# Autodesk Inventor assembly: VERSION3-largel-upright-hook
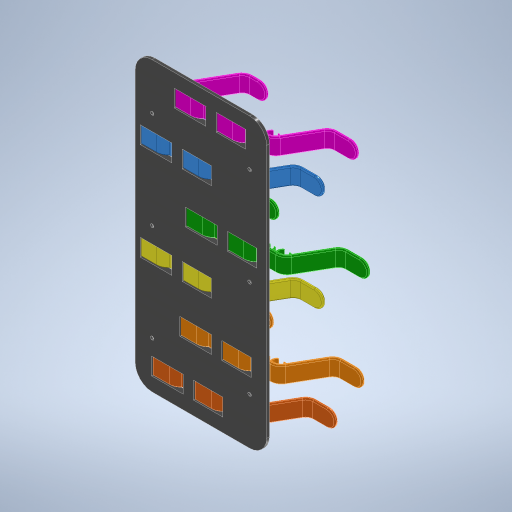
[picture p0: Inventor's stored thumbnail of the model, 512x512]
Saved by Autodesk Inventor 2024.1 (Build 281209000, 209)
## iProperties
Created: 2024-09-23
Part Number: VERSION3-largel-upright-hook
Document SubType Name: Assembly
Designer: Imogen Heard
Author: Imogen Heard
## Documents named in this file (3)
- C:\Users\iwheard\Documents\0004-CAD\3D-cad-main\cable-hanger\VERSION3-largel-upright-hook.iam
- C:\Users\iwheard\Documents\0004-CAD\3D-cad-main\cable-hanger\backplate-0.ipt
- C:\Users\iwheard\Documents\0004-CAD\3D-cad-main\cable-hanger\cable-hanger-dual-large.ipt
## Components (7 placed, 2 different names)
1. backplate-0:1 — Mate:4, Mate:5, Mate:6, Mate:7, Mate:8, Mate:9, Mate:10, Mate:11, Mate:12, Mate:13, Mate:14, Mate:15, Mate:16, Mate:17, Mate:18, Mate:19
2. cable-hanger-dual-large:1 — Mate:9
3. cable-hanger-dual-large:2 — Mate:7, Mate:13, Mate:18
4. cable-hanger-dual-large:3 — Mate:5, Mate:11, Mate:16
5. cable-hanger-dual-large:4 — Mate:8, Mate:14, Mate:19
6. cable-hanger-dual-large:5 — Mate:4, Mate:10, Mate:15
7. cable-hanger-dual-large:6 — Mate:6, Mate:12, Mate:17
## Relationships (16: Mate 16)
- Mate:4: backplate-0:1 ↔ cable-hanger-dual-large:5
- Mate:5: backplate-0:1 ↔ cable-hanger-dual-large:3
- Mate:6: backplate-0:1 ↔ cable-hanger-dual-large:6
- Mate:7: backplate-0:1 ↔ cable-hanger-dual-large:2
- Mate:8: backplate-0:1 ↔ cable-hanger-dual-large:4
- Mate:9: backplate-0:1 ↔ cable-hanger-dual-large:1
- Mate:10: backplate-0:1 ↔ cable-hanger-dual-large:5
- Mate:11: backplate-0:1 ↔ cable-hanger-dual-large:3
- Mate:12: backplate-0:1 ↔ cable-hanger-dual-large:6
- Mate:13: backplate-0:1 ↔ cable-hanger-dual-large:2
- Mate:14: backplate-0:1 ↔ cable-hanger-dual-large:4
- Mate:15: backplate-0:1 ↔ cable-hanger-dual-large:5
- Mate:16: backplate-0:1 ↔ cable-hanger-dual-large:3
- Mate:17: backplate-0:1 ↔ cable-hanger-dual-large:6
- Mate:18: backplate-0:1 ↔ cable-hanger-dual-large:2
- Mate:19: backplate-0:1 ↔ cable-hanger-dual-large:4
